# Autodesk Inventor assembly: plotter_try_2
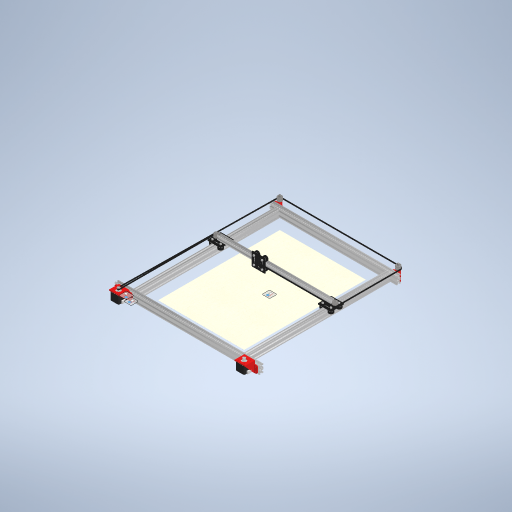
[picture p0: Inventor's stored thumbnail of the model, 512x512]
Saved by Autodesk Inventor 2023 (Build 270158000, 158)
## iProperties
RuleStatus: InUse
Created: 2023-08-15
Part Number: plotter_try_2
Document SubType Name: Assembly
Designer: Felix
_SolveAssemblyDoc: Frame Generator Solve Assembly
_Version: 15.0.0
Author: Felix
## Documents named in this file (14)
- D:\Programmieren\PineapplePenPlotter\Inventor\plotter_try_2.iam
- D:\Programmieren\PineapplePenPlotter\Inventor\PaperA2.ipt
- D:\Programmieren\PineapplePenPlotter\Inventor\plotter_try_2\Frame2.ipt
- D:\Programmieren\PineapplePenPlotter\Inventor\plotter_try_2\Frame\Frame 1692119975215.iam
- D:\Programmieren\PineapplePenPlotter\Inventor\StoreBought\4022_20220624140806_V-Slot Gantry Kit - 20mm.iam
- D:\Programmieren\PineapplePenPlotter\Inventor\plotter_try_2\YAxis.ipt
- C:\Users\Felix\Documents\Inventor\Content Center Files\R2023\en-US\BS 290 SKF(30)\BS 290 SKF - SKF 608.ipt
- D:\Programmieren\PineapplePenPlotter\Inventor\plotter_try_2\RollerHolder.ipt
- C:\Users\Felix\Documents\Inventor\Content Center Files\R2023\en-US\AS 1111\AS 1111 - M8 x 65.ipt
- D:\Programmieren\PineapplePenPlotter\Inventor\StoreBought\GT2_16T.ipt
- D:\Programmieren\PineapplePenPlotter\Inventor\steppeSquare.ipt
- D:\Programmieren\PineapplePenPlotter\Inventor\MotorBracket.ipt
- D:\Programmieren\PineapplePenPlotter\Inventor\MotorBracket - Copy.ipt
- D:\Programmieren\PineapplePenPlotter\Inventor\Belt1.ipt
## Components (26 placed, 13 different names)
1. PaperA2:1 — Flush:1, Mate:2, Angle:1, Flush:11, Flush:15
2. Frame2:1 — Flush:1
3. Frame 1692119975215:1 [sub-assembly] — Mate:1, Flush:2, Flush:3, Mate:3, Angle:2, Angle:3, Mate:8, Flush:7, Angle:4, Flush:10, Tangent:5, Mate:15, Angle:6, Angle:8, Mate:24, Mate:26
4. 4022_20220624140806_V-Slot Gantry Kit - 20mm:1 [sub-assembly] — Mate:1, Flush:2, Flush:4, Flush:5, Flush:6, Mate:4, Mate:5
5. 4022_20220624140806_V-Slot Gantry Kit - 20mm:2 [sub-assembly] — Flush:3, Mate:3, Flush:4, Mate:18, Mate:19, Mate:20
6. YAxis:1 — Flush:5, Flush:6
7. BS 290 SKF 608:1 — Mate:4, Mate:5, Mate:6, Mate:7, Flush:8, Flush:12
8. BS 290 SKF 608:2 — Mate:6, Mate:7, Tangent:1, Tangent:2, Tangent:3, Flush:9, Tangent:7, Tangent:8
9. 4022_20220624140806_V-Slot Gantry Kit - 20mm:3 [sub-assembly] — Mate:8, Flush:7
10. BS 290 SKF 608:3 — Mate:9, Flush:9, Mate:10
11. BS 290 SKF 608:4 — Tangent:4, Mate:9, Flush:8
12. AS 1111 - Metric M8 x 65:1 — Mate:10, Flush:10, Tangent:5
13. RollerHolder:1 — Flush:11, Flush:17
14. GT2_16T:1 — Tangent:6, Mate:11, Mate:14, Flush:19
15. steppeSquare:1 — Mate:11, Mate:13, Angle:5, Mate:14, Mate:15, Mate:27
16. MotorBracket:1 — Flush:15, Flush:18, Mate:27
17. BS 290 SKF 608:5 — Mate:16, Flush:16, Mate:22, Tangent:11, Mate:23
18. BS 290 SKF 608:6 — Mate:16, Tangent:9, Mate:22
19. RollerHolder:2 — Mate:23, Mate:24, Flush:17, Mate:25
20. BS 290 SKF 608:7 — Mate:19, Mate:20, Mate:21, Tangent:10
21. BS 290 SKF 608:8 — Mate:18, Mate:21, Flush:16
22. AS 1111 - Metric M8 x 65:2 — Mate:25
23. GT2_16T:2 — Tangent:12, Mate:28, Flush:20
24. MotorBracket - Copy:1 — Mate:26, Flush:18, Mate:28, Mate:29, Mate:30, Angle:9
25. Belt1:1 — Flush:19
26. steppeSquare:2 — Mate:29, Mate:30, Angle:9
## Relationships (67: Mate 28, Flush 18, Tangent 12, Angle 9)
- Flush:1: PaperA2:1 ↔ Frame2:1
- Mate:1: Frame 1692119975215:1 ↔ 4022_20220624140806_V-Slot Gantry Kit - 20mm:1
- Flush:2: Frame 1692119975215:1 ↔ 4022_20220624140806_V-Slot Gantry Kit - 20mm:1
- Mate:2: PaperA2:1
- Angle:1 (0 deg): PaperA2:1
- Flush:3: Frame 1692119975215:1 ↔ 4022_20220624140806_V-Slot Gantry Kit - 20mm:2
- Mate:3: Frame 1692119975215:1 ↔ 4022_20220624140806_V-Slot Gantry Kit - 20mm:2
- Flush:4: 4022_20220624140806_V-Slot Gantry Kit - 20mm:1 ↔ 4022_20220624140806_V-Slot Gantry Kit - 20mm:2
- Flush:5: 4022_20220624140806_V-Slot Gantry Kit - 20mm:1 ↔ YAxis:1
- Flush:6: 4022_20220624140806_V-Slot Gantry Kit - 20mm:1 ↔ YAxis:1
- Mate:4 (2 mm): 4022_20220624140806_V-Slot Gantry Kit - 20mm:1 ↔ BS 290 SKF 608:1
- Mate:5: 4022_20220624140806_V-Slot Gantry Kit - 20mm:1 ↔ BS 290 SKF 608:1
- Mate:6 (2 mm): BS 290 SKF 608:1 ↔ BS 290 SKF 608:2
- Mate:7: BS 290 SKF 608:1 ↔ BS 290 SKF 608:2
- Angle:2 (0 deg): Frame 1692119975215:1
- Tangent:1: BS 290 SKF 608:2
- Angle:3 (0 deg): Frame 1692119975215:1
- Tangent:2: BS 290 SKF 608:2
- Mate:8: Frame 1692119975215:1 ↔ 4022_20220624140806_V-Slot Gantry Kit - 20mm:3
- Flush:7: Frame 1692119975215:1 ↔ 4022_20220624140806_V-Slot Gantry Kit - 20mm:3
- Angle:4 (0 deg): Frame 1692119975215:1
- Tangent:3: BS 290 SKF 608:2
- Tangent:4: BS 290 SKF 608:4
- Mate:9: BS 290 SKF 608:3 ↔ BS 290 SKF 608:4
- Flush:8: BS 290 SKF 608:1 ↔ BS 290 SKF 608:4
- Flush:9: BS 290 SKF 608:2 ↔ BS 290 SKF 608:3
- Mate:10: BS 290 SKF 608:3 ↔ AS 1111 - Metric M8 x 65:1
- Flush:10: Frame 1692119975215:1 ↔ AS 1111 - Metric M8 x 65:1
- Tangent:5 (5 mm): Frame 1692119975215:1 ↔ AS 1111 - Metric M8 x 65:1
- Flush:11: PaperA2:1 ↔ RollerHolder:1
- Flush:12 (-3.5 mm): BS 290 SKF 608:1
- Tangent:6 (1.3 mm): GT2_16T:1
- Mate:11: GT2_16T:1 ↔ steppeSquare:1
- Mate:13: steppeSquare:1
- Angle:5 (0 deg): steppeSquare:1
- Mate:14 (0.5 mm): GT2_16T:1 ↔ steppeSquare:1
- Mate:15 (5.5 mm): Frame 1692119975215:1 ↔ steppeSquare:1
- Flush:15: PaperA2:1 ↔ MotorBracket:1
- Angle:6 (0 deg): Frame 1692119975215:1
- Tangent:7: BS 290 SKF 608:2
- Angle:7 (0 deg)
- Tangent:8: BS 290 SKF 608:2
- Mate:16: BS 290 SKF 608:5 ↔ BS 290 SKF 608:6
- Tangent:9: BS 290 SKF 608:6
- Mate:18: 4022_20220624140806_V-Slot Gantry Kit - 20mm:2 ↔ BS 290 SKF 608:8
- Mate:19: 4022_20220624140806_V-Slot Gantry Kit - 20mm:2 ↔ BS 290 SKF 608:7
- Mate:20 (2 mm): 4022_20220624140806_V-Slot Gantry Kit - 20mm:2 ↔ BS 290 SKF 608:7
- Mate:21 (2 mm): BS 290 SKF 608:7 ↔ BS 290 SKF 608:8
- Flush:16: BS 290 SKF 608:5 ↔ BS 290 SKF 608:8
- Mate:22 (2 mm): BS 290 SKF 608:5 ↔ BS 290 SKF 608:6
- Angle:8 (0 deg): Frame 1692119975215:1
- Tangent:10: BS 290 SKF 608:7
- Tangent:11: BS 290 SKF 608:5
- Mate:23: BS 290 SKF 608:5 ↔ RollerHolder:2
- Mate:24: Frame 1692119975215:1 ↔ RollerHolder:2
- Flush:17: RollerHolder:1 ↔ RollerHolder:2
- Mate:25: RollerHolder:2 ↔ AS 1111 - Metric M8 x 65:2
- Mate:26: Frame 1692119975215:1 ↔ MotorBracket - Copy:1
- Flush:18: MotorBracket:1 ↔ MotorBracket - Copy:1
- Mate:27: steppeSquare:1 ↔ MotorBracket:1
- Tangent:12 (1.3 mm): GT2_16T:2
- Mate:28: GT2_16T:2 ↔ MotorBracket - Copy:1
- Flush:19: GT2_16T:1 ↔ Belt1:1
- Flush:20 (54.95 mm): GT2_16T:2
- Mate:29: MotorBracket - Copy:1 ↔ steppeSquare:2
- Mate:30: MotorBracket - Copy:1 ↔ steppeSquare:2
- Angle:9 (0 deg): MotorBracket - Copy:1 ↔ steppeSquare:2
## Named parameters: ROLLER_SPACING = 2 mm, BELT_THICKNESS = 1.5 mm, RIGHT_MOTOR_HEIGHT = 50 mm
